# Autodesk Inventor assembly: A2017_T5_01
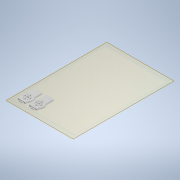
[picture p0: Inventor's stored thumbnail of the model, 180x180]
Saved by Autodesk Inventor 2020 (Build 240168000, 168)
## iProperties
Created: 2021-08-27
Part Number: A2017_T5_01
Document SubType Name: Assembly
Designer: Masato
Author: Masato
## Documents named in this file (3)
- C:\Users\L20C1118 森　圭汰\Documents\220111_openplatform\OpenPlatform_ver3_0\cam\A2017_T5_01.iam
- C:\Users\L20C1118 森　圭汰\Documents\220111_openplatform\OpenPlatform_ver3_0\cam\Disposable_Board.ipt
- C:\Users\L20C1118 森　圭汰\Documents\220111_openplatform\OpenPlatform_ver3_0\LowerBody\Leg_joit\Leg_joint_yaw_frame.ipt
## Components (3 placed, 2 different names)
1. Disposable_Board:1 — メイト:2, メイト:1, フラッシュ:1, フラッシュ:2, フラッシュ:3, 正接:1
2. Leg_joint_yaw_frame:1 — メイト:4, フラッシュ:3, 正接:1, フラッシュ:4, 正接:2, フラッシュ:5
3. Leg_joint_yaw_frame:2 — フラッシュ:4, 正接:2, フラッシュ:5, メイト:5
## Relationships (11: Flush 5, Mate 4, Tangent 2)
- メイト:2 [Mate]: Disposable_Board:1
- メイト:1 [Mate]: Disposable_Board:1
- フラッシュ:1 [Flush]: Disposable_Board:1
- フラッシュ:2 [Flush]: Disposable_Board:1
- メイト:4 [Mate]: Leg_joint_yaw_frame:1
- フラッシュ:3 [Flush] (3 mm): Disposable_Board:1 ↔ Leg_joint_yaw_frame:1
- 正接:1 [Tangent] (3 mm): Disposable_Board:1 ↔ Leg_joint_yaw_frame:1
- フラッシュ:4 [Flush]: Leg_joint_yaw_frame:1 ↔ Leg_joint_yaw_frame:2
- 正接:2 [Tangent] (3 mm): Leg_joint_yaw_frame:1 ↔ Leg_joint_yaw_frame:2
- フラッシュ:5 [Flush]: Leg_joint_yaw_frame:1 ↔ Leg_joint_yaw_frame:2
- メイト:5 [Mate]: Leg_joint_yaw_frame:2
